# Autodesk Inventor assembly: Battery_Holder_Assembly
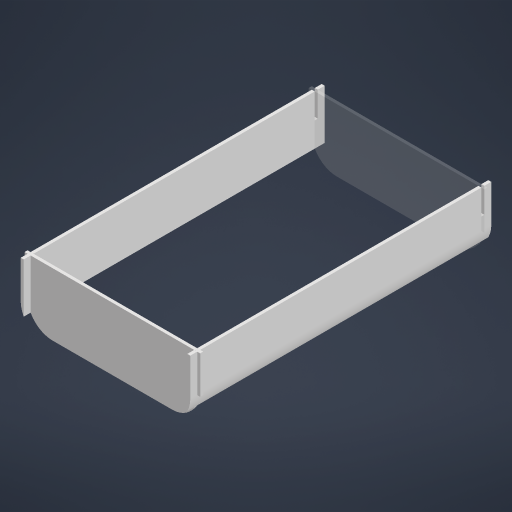
[picture p0: Inventor's stored thumbnail of the model, 512x512]
Saved by Autodesk Inventor 2024 (Build 280153000, 153)
## iProperties
Created: 2024-02-28
Part Number: Battery_Holder_Assembly
Document SubType Name: Assembly
Designer: calvi
Author: calvi
## Documents named in this file (3)
- C:\Users\calvi\OneDrive\Robocup Rescue\Chassis\Battery Drawer\BatteryHolder\Battery_Holder_Assembly.iam
- C:\Users\calvi\OneDrive\Robocup Rescue\Chassis\Battery Drawer\BatteryHolder\Battery_container_main.ipt
- C:\Users\calvi\OneDrive\Robocup Rescue\Chassis\Battery Drawer\BatteryHolder\Battery_container_side.ipt
## Components (4 placed, 2 different names)
1. Battery_container_main:1 — Mate:8, Mate:9, Mate:10
2. Battery_container_main:2 — Mate:1, Mate:2, Mate:3, Mate:4, Mate:5, Mate:6
3. Battery_container_side:2 — Mate:1, Mate:2, Mate:3
4. Battery_container_side:3 — Mate:4, Mate:5, Mate:6, Mate:8, Mate:9, Mate:10
## Relationships (9: Mate 9)
- Mate:1: Battery_container_main:2 ↔ Battery_container_side:2
- Mate:2: Battery_container_main:2 ↔ Battery_container_side:2
- Mate:3: Battery_container_main:2 ↔ Battery_container_side:2
- Mate:4: Battery_container_main:2 ↔ Battery_container_side:3
- Mate:5: Battery_container_main:2 ↔ Battery_container_side:3
- Mate:6: Battery_container_main:2 ↔ Battery_container_side:3
- Mate:8: Battery_container_main:1 ↔ Battery_container_side:3
- Mate:9: Battery_container_main:1 ↔ Battery_container_side:3
- Mate:10: Battery_container_main:1 ↔ Battery_container_side:3
